# Autodesk Inventor assembly: Chassis-ver18-1111-2019
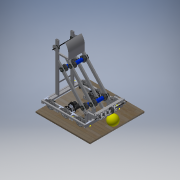
[picture p0: Inventor's stored thumbnail of the model, 180x180]
Saved by Autodesk Inventor 2018 (Build 220112000, 112)
## iProperties
Created: 2019-10-10
Part Number: Chassis-ver18-1111-2019
Document SubType Name: Assembly
Designer: JMHal
Author: JMHal
## Documents named in this file (21)
- F:\GrabCad\2020 Infinite Recharge\Chassis\Assembly\Chassis-ver18-1111-2019.iam
- F:\GrabCad\2020 Infinite Recharge\Chassis\Parts\2x1 20in Alluminum with Cal Drop.ver1-1111-2019.ipt
- F:\GrabCad\2020 Infinite Recharge\Chassis\Parts\2x1 20in Alluminum.ver1-1111-2019.ipt
- F:\GrabCad\2020 Infinite Recharge\Chassis\Parts\2x1 2in Alluminum Block.ver1-1111-2019.ipt
- F:\GrabCad\Resources\VEXpro Resources\Bearings\0.5inHexFlangedBearing(1.125inx0.313in)-1111-2016.ipt
- F:\GrabCad\Resources\VEXpro Resources\Versa Motion\VersaBlockKit-1111-2016.ipt
- F:\GrabCad\Resources\VEXpro Resources\Gearboxes\WCP SS Gearbox\SS-Gearbox.iam
- F:\GrabCad\Resources\VEXpro Resources\Gussets\ChassisGusset-1111-2016.ipt
- F:\GrabCad\Resources\VEXpro Resources\Wheels\6 inch\6x1inTractionWheel-1111-2016.iam
- F:\GrabCad\2020 Infinite Recharge\Chassis\Parts\Bumbers.ver1-1111-2019.ipt
- F:\GrabCad\Season Archives\2019 - Deep Space\Chassis\Parts\AluminumBracket.ipt
- F:\GrabCad\2020 Infinite Recharge\Chassis\Parts\BumperMount1-ver1-1111-2019.ipt
- F:\GrabCad\2020 Infinite Recharge\Intake\Assemblies\IntakeAssembly-ver1-1111-2020.iam
- F:\GrabCad\2020 Infinite Recharge\Platform.ver1-1111-2020.ipt
- F:\GrabCad\2020 Infinite Recharge\Powercell.ver1-1111-2020.ipt
- F:\GrabCad\2020 Infinite Recharge\Shooting\Assemblies\ShooterPrototype-ver2-1111-2019.iam
- F:\GrabCad\2020 Infinite Recharge\Storage\Assemblies\StorageAssembly.ver4-1111-2020.iam
- F:\GrabCad\2020 Infinite Recharge\Chassis\Parts\ElectricalBoard.ver2-1111-2020.ipt
- F:\GrabCad\Resources\VEXpro Resources\Shafts\0.5inThunderHexShaft(8)-1111-2016_MIR.ipt
- F:\GrabCad\Resources\VEXpro Resources\Shafts\0.5inThunderHexShaft(5in(modified))-1111-2016.ipt
- F:\GrabCad\2020 Infinite Recharge\Integration\Assemblies\Roller-ver1-1111-2019.iam
## Components (101 placed, 20 different names)
1. 2x1 20in Alluminum with Cal Drop.ver1-1111-2019:1 — Mate:31, Mate:32, Insert:8, Mate:53, Angle:9, Insert:19, Angle:11, Flush:1, Mate:65, Mate:66, Flush:2, Mate:67, Flush:4, Flush:5, Mate:77, Mate:78, Flush:16, Flush:17, Mate:80, Flush:20, Flush:23, Symmetry:1, Symmetry:2, Flush:62, Mate:141, Mate:146, Angle:15, Mate:147, Mate:148, Angle:16, Mate:149, Cylindrical:65, Mate:209, Angle:23, Mate:215, Flush:66, Mate:219, Flush:69
2. 2x1 20in Alluminum.ver1-1111-2019:1 — Mate:65, Mate:66, Flush:2, Mate:68, Mate:72, Mate:81, Flush:22, Mate:82, Flush:24, Flush:62, Mate:140, Flush:63, Mate:197, Mate:198, Mate:199, Mate:200, Mate:201, Mate:212
3. 2x1 20in Alluminum with Cal Drop.ver1-1111-2019:2 — Insert:5, Angle:7, Insert:23, Angle:13, Flush:6, Flush:8, Mate:73, Flush:9, Flush:34, Flush:35, Flush:36, Flush:37, Symmetry:1, Symmetry:2, Mate:142, Mate:143, Mate:156, Mate:157, Angle:17, Mate:158, Mate:159, Angle:18, Cylindrical:64, Mate:208, Angle:22, Mate:211, Flush:64, Flush:65
4. 2x1 20in Alluminum.ver1-1111-2019:2 — Mate:67, Flush:4, Flush:5, Mate:69, Flush:6, Mate:71, Mate:73, Mate:79, Flush:19, Flush:21, Mate:214, Flush:68
5. ChassisGusset-1111-2016:1 — Mate:76, Flush:12, Flush:36
6. ChassisGusset-1111-2016:2 — Mate:75, Flush:11, Flush:35
7. ChassisGusset-1111-2016:3 — Mate:78, Flush:14, Flush:17
8. ChassisGusset-1111-2016:4 — Mate:77, Flush:15, Flush:16
9. ChassisGusset-1111-2016:5 — Mate:82, Flush:24, Flush:34
10. ChassisGusset-1111-2016:6 — Mate:81, Flush:22, Flush:23
11. ChassisGusset-1111-2016:7 — Mate:80, Flush:20, Flush:21
12. ChassisGusset-1111-2016:8 — Mate:79, Flush:19, Flush:37, Mate:216
13. 6x1inTractionWheel-1111-2016:5 [sub-assembly] — Cylindrical:68, Mate:220
14. Bumbers.ver1-1111-2019:1 — Mate:139, Mate:140, Mate:210
15. VersaBlockKit-1111-2016:13 — Mate:146, Angle:15, Mate:147, Rotational:17
16. VersaBlockKit-1111-2016:14 — Mate:148, Angle:16, Mate:149, Cylindrical:45, Mate:153, Cylindrical:122, Mate:291
17. 0.5inHexFlangedBearing(1.125inx0.313in)-1111-2016:21 — Cylindrical:45, Mate:153
18. 6x1inTractionWheel-1111-2016:11 [sub-assembly] — Cylindrical:123, Mate:291
19. 0.5inHexFlangedBearing(1.125inx0.313in)-1111-2016:22 — Rotational:17
20. VersaBlockKit-1111-2016:15 — Mate:156, Mate:157, Angle:17, Mate:160, Angle:19, Mate:290
21. VersaBlockKit-1111-2016:16 — Mate:158, Mate:159, Angle:18, Mate:161, Mate:165, Angle:21
22. 0.5inHexFlangedBearing(1.125inx0.313in)-1111-2016:23 — Mate:160, Angle:19, Cylindrical:120
23. 0.5inHexFlangedBearing(1.125inx0.313in)-1111-2016:24 — Mate:161, Mate:165, Angle:21
24. 6x1inTractionWheel-1111-2016:12 [sub-assembly] — Cylindrical:121, Mate:290
25. 6x1inTractionWheel-1111-2016:13 [sub-assembly] — Cylindrical:124, Mate:292
26. 6x1inTractionWheel-1111-2016:14 [sub-assembly] — Cylindrical:69, Mate:221
27. AluminumBracket:1 — Mate:167, Mate:168, Mate:169
28. AluminumBracket:4 — Mate:176, Mate:177, Mate:178
29. AluminumBracket:5 — Mate:179, Mate:180, Mate:181
30. AluminumBracket:7 — Mate:185, Mate:186, Mate:187
31. BumperMount1-ver1-1111-2019:2 — Mate:197, Mate:198, Mate:199, Mate:210
32. BumperMount1-ver1-1111-2019:3 — Mate:200, Mate:201
33. SS-Gearbox:1 [sub-assembly] — Cylindrical:65, Mate:209, Angle:23, Cylindrical:124, Mate:292
34. SS-Gearbox:2 [sub-assembly] — Cylindrical:64, Mate:208, Angle:22, Cylindrical:69, Mate:221
35. IntakeAssembly-ver1-1111-2020:1 [sub-assembly] — Mate:211, Flush:64, Mate:212
36. Platform.ver1-1111-2020:1 — Flush:65, Mate:214, Tangent:2
37. Powercell.ver1-1111-2020:1 — Tangent:2
38. ShooterPrototype-ver2-1111-2019:1 [sub-assembly] — Mate:215, Flush:66, Mate:216, Mate:217, Flush:67, Mate:218
39. StorageAssembly.ver4-1111-2020:1 [sub-assembly] — Mate:217, Flush:67, Mate:218, Mate:234, Mate:235, Angle:24, Mate:237, Mate:238, Angle:25, Mate:241, Mate:242, Angle:26, Mate:243, Mate:244, Angle:27, Cylindrical:92, Mate:248, Mate:249, Angle:28, Mate:250, Mate:251, Angle:29, Mate:252, Mate:253, Angle:30, Mate:254, Mate:255, Angle:31, Mate:262, Mate:263, Angle:32, Mate:264, Mate:265, Angle:33, Mate:266, Mate:267, Angle:34, Mate:268, Mate:269, Angle:35, Mate:270, Mate:271, Angle:36, Mate:272, Mate:273, Angle:37, Mate:274, Mate:275, Angle:38, Mate:276, Mate:277, Angle:39
40. ElectricalBoard.ver2-1111-2020:1 — Mate:219, Flush:68, Flush:69
41. 0.5inThunderHexShaft(8)-1111-2016_MIR:1 — Cylindrical:67, Cylindrical:68
42. 0.5inThunderHexShaft(8)-1111-2016_MIR:2 — Cylindrical:120, Cylindrical:121
43. 0.5inHexFlangedBearing(1.125inx0.313in)-1111-2016:25 — Cylindrical:88, Mate:236, Flush:72
44. 0.5inHexFlangedBearing(1.125inx0.313in)-1111-2016:27 — Cylindrical:89, Mate:239, Cylindrical:90
45. 0.5inThunderHexShaft(5in(modified))-1111-2016:1 — Cylindrical:90, Flush:72
46. VersaBlockKit-1111-2016:17 — Mate:234, Mate:235, Angle:24, Cylindrical:88, Mate:236
47. VersaBlockKit-1111-2016:18 — Mate:237, Mate:238, Angle:25, Cylindrical:89, Mate:239
48. VersaBlockKit-1111-2016:19 — Mate:241, Mate:242, Angle:26, Mate:245
49. VersaBlockKit-1111-2016:20 — Mate:243, Mate:244, Angle:27, Cylindrical:93, Mate:246
50. 0.5inHexFlangedBearing(1.125inx0.313in)-1111-2016:33 — Cylindrical:92, Mate:245, Flush:73
51. 0.5inHexFlangedBearing(1.125inx0.313in)-1111-2016:34 — Cylindrical:93, Mate:246, Cylindrical:94
52. 0.5inThunderHexShaft(5in(modified))-1111-2016:5 — Cylindrical:94, Flush:73
53. VersaBlockKit-1111-2016:21 — Mate:248, Mate:249, Angle:28, Cylindrical:97, Mate:257
54. VersaBlockKit-1111-2016:22 — Mate:250, Mate:251, Angle:29, Cylindrical:96, Mate:256
55. VersaBlockKit-1111-2016:23 — Mate:252, Mate:253, Angle:30, Cylindrical:98, Mate:258
56. VersaBlockKit-1111-2016:24 — Mate:254, Mate:255, Angle:31, Cylindrical:99, Mate:259
57. 0.5inHexFlangedBearing(1.125inx0.313in)-1111-2016:35 — Cylindrical:96, Mate:256, Flush:70
58. 0.5inHexFlangedBearing(1.125inx0.313in)-1111-2016:36 — Cylindrical:97, Mate:257, Flush:71
59. 0.5inHexFlangedBearing(1.125inx0.313in)-1111-2016:37 — Cylindrical:98, Mate:258, Cylindrical:101
60. 0.5inHexFlangedBearing(1.125inx0.313in)-1111-2016:38 — Cylindrical:99, Mate:259, Cylindrical:100
61. 0.5inThunderHexShaft(5in(modified))-1111-2016:6 — Cylindrical:100, Flush:70
62. 0.5inThunderHexShaft(5in(modified))-1111-2016:7 — Cylindrical:101, Flush:71
63. VersaBlockKit-1111-2016:25 — Mate:262, Mate:263, Angle:32, Cylindrical:104, Mate:278
64. VersaBlockKit-1111-2016:26 — Mate:264, Mate:265, Angle:33, Cylindrical:105, Mate:279
65. VersaBlockKit-1111-2016:27 — Mate:266, Mate:267, Angle:34, Cylindrical:111, Mate:285
66. VersaBlockKit-1111-2016:28 — Mate:268, Mate:269, Angle:35, Cylindrical:109, Mate:283
67. VersaBlockKit-1111-2016:29 — Mate:270, Mate:271, Angle:36, Cylindrical:110, Mate:284
68. VersaBlockKit-1111-2016:30 — Mate:272, Mate:273, Angle:37, Cylindrical:108, Mate:282
69. VersaBlockKit-1111-2016:31 — Mate:274, Mate:275, Angle:38, Cylindrical:106, Mate:280
70. VersaBlockKit-1111-2016:32 — Mate:276, Mate:277, Angle:39, Cylindrical:107, Mate:281
71. 0.5inHexFlangedBearing(1.125inx0.313in)-1111-2016:39 — Cylindrical:104, Mate:278, Cylindrical:113, Flush:76
72. 0.5inHexFlangedBearing(1.125inx0.313in)-1111-2016:40 — Cylindrical:105, Mate:279, Cylindrical:115, Flush:75
73. 0.5inHexFlangedBearing(1.125inx0.313in)-1111-2016:41 — Cylindrical:106, Mate:280, Cylindrical:114, Flush:77
74. 0.5inHexFlangedBearing(1.125inx0.313in)-1111-2016:42 — Cylindrical:107, Mate:281, Cylindrical:112, Flush:74
75. 0.5inHexFlangedBearing(1.125inx0.313in)-1111-2016:43 — Cylindrical:108, Mate:282, Mate:305
76. 0.5inHexFlangedBearing(1.125inx0.313in)-1111-2016:44 — Cylindrical:109, Mate:283, Mate:306
77. 0.5inHexFlangedBearing(1.125inx0.313in)-1111-2016:45 — Cylindrical:110, Mate:284, Mate:307
78. 0.5inHexFlangedBearing(1.125inx0.313in)-1111-2016:46 — Cylindrical:111, Mate:285, Mate:308
79. 0.5inThunderHexShaft(5in(modified))-1111-2016:8 — Cylindrical:112, Cylindrical:138, Flush:74
80. 0.5inThunderHexShaft(5in(modified))-1111-2016:9 — Cylindrical:113, Cylindrical:137, Flush:76
81. 0.5inThunderHexShaft(5in(modified))-1111-2016:10 — Cylindrical:114, Cylindrical:136, Flush:77
82. 0.5inThunderHexShaft(5in(modified))-1111-2016:11 — Cylindrical:115, Cylindrical:139, Flush:75
83. 0.5inThunderHexShaft(8)-1111-2016_MIR:3 — Cylindrical:122, Cylindrical:123
84. 0.5inThunderHexShaft(8)-1111-2016_MIR:4 — Cylindrical:125, Cylindrical:126
85. 6x1inTractionWheel-1111-2016:15 [sub-assembly] — Cylindrical:126, Mate:293
86. Roller-ver1-1111-2019:1 [sub-assembly] — Cylindrical:136, Mate:305
87. Roller-ver1-1111-2019:2 [sub-assembly] — Cylindrical:137, Mate:306
88. Roller-ver1-1111-2019:3 [sub-assembly] — Cylindrical:138, Mate:307
89. Roller-ver1-1111-2019:4 [sub-assembly] — Cylindrical:139, Mate:308
90. 0.5inHexFlangedBearing(1.125inx0.313in)-1111-2016:19
91. 0.5inHexFlangedBearing(1.125inx0.313in)-1111-2016:7 — Insert:5, Mate:48, Mate:49
92. 0.5inHexFlangedBearing(1.125inx0.313in)-1111-2016:17 — Insert:19
93. 0.5inHexFlangedBearing(1.125inx0.313in)-1111-2016:10 — Insert:8, Mate:52, Cylindrical:125
94. 2x1 2in Alluminum Block.ver1-1111-2019:5 — Mate:31, Mate:32, Mate:69, Flush:15, Mate:167, Mate:168, Mate:169
95. 2x1 2in Alluminum Block.ver1-1111-2019:6 — Flush:1, Mate:68, Flush:14, Mate:141, Mate:176, Mate:177, Mate:178
96. 2x1 2in Alluminum Block.ver1-1111-2019:7 — Mate:72, Flush:9, Mate:75, Flush:11, Mate:143, Flush:63, Mate:179, Mate:180, Mate:181
97. 2x1 2in Alluminum Block.ver1-1111-2019:8 — Flush:8, Mate:71, Mate:76, Flush:12, Mate:139, Mate:142, Mate:185, Mate:186, Mate:187
98. VersaBlockKit-1111-2016:3 — Mate:48, Mate:49, Angle:7, Cylindrical:67, Mate:220
99. VersaBlockKit-1111-2016:6 — Mate:52, Mate:53, Angle:9, Mate:293
100. VersaBlockKit-1111-2016:9 — Angle:11
101. VersaBlockKit-1111-2016:11 — Insert:23, Angle:13
## Relationships (245: Mate 127, CylindricalJoint 41, Flush 39, Angle 28, Insert 6, Symmetry 2, RevoluteJoint 1, Tangent 1)
- Mate:31: 2x1 20in Alluminum with Cal Drop.ver1-1111-2019:1 ↔ 2x1 2in Alluminum Block.ver1-1111-2019:5
- Mate:32: 2x1 20in Alluminum with Cal Drop.ver1-1111-2019:1 ↔ 2x1 2in Alluminum Block.ver1-1111-2019:5
- Insert:5: 2x1 20in Alluminum with Cal Drop.ver1-1111-2019:2 ↔ 0.5inHexFlangedBearing(1.125inx0.313in)-1111-2016:7
- Mate:48: 0.5inHexFlangedBearing(1.125inx0.313in)-1111-2016:7 ↔ VersaBlockKit-1111-2016:3
- Mate:49: 0.5inHexFlangedBearing(1.125inx0.313in)-1111-2016:7 ↔ VersaBlockKit-1111-2016:3
- Insert:8: 2x1 20in Alluminum with Cal Drop.ver1-1111-2019:1 ↔ 0.5inHexFlangedBearing(1.125inx0.313in)-1111-2016:10
- Angle:7 (0 deg): 2x1 20in Alluminum with Cal Drop.ver1-1111-2019:2 ↔ VersaBlockKit-1111-2016:3
- Mate:52: 0.5inHexFlangedBearing(1.125inx0.313in)-1111-2016:10 ↔ VersaBlockKit-1111-2016:6
- Mate:53: 2x1 20in Alluminum with Cal Drop.ver1-1111-2019:1 ↔ VersaBlockKit-1111-2016:6
- Angle:9 (0 deg): 2x1 20in Alluminum with Cal Drop.ver1-1111-2019:1 ↔ VersaBlockKit-1111-2016:6
- [Mate]: 0.5inHexFlangedBearing(1.125inx0.313in)-1111-2016:17 ↔ VersaBlockKit-1111-2016:9
- [Insert]: 0.5inHexFlangedBearing(1.125inx0.313in)-1111-2016:17 ↔ VersaBlockKit-1111-2016:9
- Insert:19: 2x1 20in Alluminum with Cal Drop.ver1-1111-2019:1 ↔ 0.5inHexFlangedBearing(1.125inx0.313in)-1111-2016:17
- Angle:11 (0 deg): 2x1 20in Alluminum with Cal Drop.ver1-1111-2019:1 ↔ VersaBlockKit-1111-2016:9
- [Mate]: 0.5inHexFlangedBearing(1.125inx0.313in)-1111-2016:19 ↔ VersaBlockKit-1111-2016:11
- [Insert]: 0.5inHexFlangedBearing(1.125inx0.313in)-1111-2016:19 ↔ VersaBlockKit-1111-2016:11
- Insert:23: 2x1 20in Alluminum with Cal Drop.ver1-1111-2019:2 ↔ VersaBlockKit-1111-2016:11
- Angle:13 (0 deg): 2x1 20in Alluminum with Cal Drop.ver1-1111-2019:2 ↔ VersaBlockKit-1111-2016:11
- Flush:1: 2x1 20in Alluminum with Cal Drop.ver1-1111-2019:1 ↔ 2x1 2in Alluminum Block.ver1-1111-2019:6
- Mate:65: 2x1 20in Alluminum with Cal Drop.ver1-1111-2019:1 ↔ 2x1 20in Alluminum.ver1-1111-2019:1
- Mate:66: 2x1 20in Alluminum with Cal Drop.ver1-1111-2019:1 ↔ 2x1 20in Alluminum.ver1-1111-2019:1
- Flush:2: 2x1 20in Alluminum with Cal Drop.ver1-1111-2019:1 ↔ 2x1 20in Alluminum.ver1-1111-2019:1
- Mate:67: 2x1 20in Alluminum with Cal Drop.ver1-1111-2019:1 ↔ 2x1 20in Alluminum.ver1-1111-2019:2
- Flush:4: 2x1 20in Alluminum with Cal Drop.ver1-1111-2019:1 ↔ 2x1 20in Alluminum.ver1-1111-2019:2
- Flush:5 (-69.85 mm): 2x1 20in Alluminum with Cal Drop.ver1-1111-2019:1 ↔ 2x1 20in Alluminum.ver1-1111-2019:2
- Mate:68 (254 mm): 2x1 20in Alluminum.ver1-1111-2019:1 ↔ 2x1 2in Alluminum Block.ver1-1111-2019:6
- Mate:69 (254 mm): 2x1 20in Alluminum.ver1-1111-2019:2 ↔ 2x1 2in Alluminum Block.ver1-1111-2019:5
- Flush:6: 2x1 20in Alluminum with Cal Drop.ver1-1111-2019:2 ↔ 2x1 20in Alluminum.ver1-1111-2019:2
- Flush:8: 2x1 20in Alluminum with Cal Drop.ver1-1111-2019:2 ↔ 2x1 2in Alluminum Block.ver1-1111-2019:8
- Mate:71 (254 mm): 2x1 20in Alluminum.ver1-1111-2019:2 ↔ 2x1 2in Alluminum Block.ver1-1111-2019:8
- Mate:72 (254 mm): 2x1 20in Alluminum.ver1-1111-2019:1 ↔ 2x1 2in Alluminum Block.ver1-1111-2019:7
- Mate:73: 2x1 20in Alluminum with Cal Drop.ver1-1111-2019:2 ↔ 2x1 20in Alluminum.ver1-1111-2019:2
- Flush:9: 2x1 20in Alluminum with Cal Drop.ver1-1111-2019:2 ↔ 2x1 2in Alluminum Block.ver1-1111-2019:7
- Mate:75: ChassisGusset-1111-2016:2 ↔ 2x1 2in Alluminum Block.ver1-1111-2019:7
- Flush:11: ChassisGusset-1111-2016:2 ↔ 2x1 2in Alluminum Block.ver1-1111-2019:7
- Mate:76: ChassisGusset-1111-2016:1 ↔ 2x1 2in Alluminum Block.ver1-1111-2019:8
- Flush:12: ChassisGusset-1111-2016:1 ↔ 2x1 2in Alluminum Block.ver1-1111-2019:8
- Mate:77: 2x1 20in Alluminum with Cal Drop.ver1-1111-2019:1 ↔ ChassisGusset-1111-2016:4
- Mate:78: 2x1 20in Alluminum with Cal Drop.ver1-1111-2019:1 ↔ ChassisGusset-1111-2016:3
- Flush:14: ChassisGusset-1111-2016:3 ↔ 2x1 2in Alluminum Block.ver1-1111-2019:6
- Flush:15: ChassisGusset-1111-2016:4 ↔ 2x1 2in Alluminum Block.ver1-1111-2019:5
- Flush:16: 2x1 20in Alluminum with Cal Drop.ver1-1111-2019:1 ↔ ChassisGusset-1111-2016:4
- Flush:17: 2x1 20in Alluminum with Cal Drop.ver1-1111-2019:1 ↔ ChassisGusset-1111-2016:3
- Mate:79: 2x1 20in Alluminum.ver1-1111-2019:2 ↔ ChassisGusset-1111-2016:8
- Flush:19: 2x1 20in Alluminum.ver1-1111-2019:2 ↔ ChassisGusset-1111-2016:8
- Mate:80: 2x1 20in Alluminum with Cal Drop.ver1-1111-2019:1 ↔ ChassisGusset-1111-2016:7
- Flush:20: 2x1 20in Alluminum with Cal Drop.ver1-1111-2019:1 ↔ ChassisGusset-1111-2016:7
- Flush:21: 2x1 20in Alluminum.ver1-1111-2019:2 ↔ ChassisGusset-1111-2016:7
- Mate:81: 2x1 20in Alluminum.ver1-1111-2019:1 ↔ ChassisGusset-1111-2016:6
- Flush:22: 2x1 20in Alluminum.ver1-1111-2019:1 ↔ ChassisGusset-1111-2016:6
- Flush:23: 2x1 20in Alluminum with Cal Drop.ver1-1111-2019:1 ↔ ChassisGusset-1111-2016:6
- Mate:82: 2x1 20in Alluminum.ver1-1111-2019:1 ↔ ChassisGusset-1111-2016:5
- Flush:24: 2x1 20in Alluminum.ver1-1111-2019:1 ↔ ChassisGusset-1111-2016:5
- Flush:34: 2x1 20in Alluminum with Cal Drop.ver1-1111-2019:2 ↔ ChassisGusset-1111-2016:5
- Flush:35: 2x1 20in Alluminum with Cal Drop.ver1-1111-2019:2 ↔ ChassisGusset-1111-2016:2
- Flush:36: 2x1 20in Alluminum with Cal Drop.ver1-1111-2019:2 ↔ ChassisGusset-1111-2016:1
- Flush:37: 2x1 20in Alluminum with Cal Drop.ver1-1111-2019:2 ↔ ChassisGusset-1111-2016:8
- Symmetry:1: 2x1 20in Alluminum with Cal Drop.ver1-1111-2019:1 ↔ 2x1 20in Alluminum with Cal Drop.ver1-1111-2019:2
- Symmetry:2: 2x1 20in Alluminum with Cal Drop.ver1-1111-2019:1 ↔ 2x1 20in Alluminum with Cal Drop.ver1-1111-2019:2
- Flush:62 (69.85 mm): 2x1 20in Alluminum with Cal Drop.ver1-1111-2019:1 ↔ 2x1 20in Alluminum.ver1-1111-2019:1
- Mate:139 (-127 mm): Bumbers.ver1-1111-2019:1 ↔ 2x1 2in Alluminum Block.ver1-1111-2019:8
- Mate:140: 2x1 20in Alluminum.ver1-1111-2019:1 ↔ Bumbers.ver1-1111-2019:1
- Mate:141: 2x1 20in Alluminum with Cal Drop.ver1-1111-2019:1 ↔ 2x1 2in Alluminum Block.ver1-1111-2019:6
- Mate:142: 2x1 20in Alluminum with Cal Drop.ver1-1111-2019:2 ↔ 2x1 2in Alluminum Block.ver1-1111-2019:8
- Mate:143: 2x1 20in Alluminum with Cal Drop.ver1-1111-2019:2 ↔ 2x1 2in Alluminum Block.ver1-1111-2019:7
- Flush:63: 2x1 20in Alluminum.ver1-1111-2019:1 ↔ 2x1 2in Alluminum Block.ver1-1111-2019:7
- Mate:146: 2x1 20in Alluminum with Cal Drop.ver1-1111-2019:1 ↔ VersaBlockKit-1111-2016:13
- Angle:15 (0 deg): 2x1 20in Alluminum with Cal Drop.ver1-1111-2019:1 ↔ VersaBlockKit-1111-2016:13
- Mate:147: 2x1 20in Alluminum with Cal Drop.ver1-1111-2019:1 ↔ VersaBlockKit-1111-2016:13
- Mate:148: 2x1 20in Alluminum with Cal Drop.ver1-1111-2019:1 ↔ VersaBlockKit-1111-2016:14
- Angle:16 (0 deg): 2x1 20in Alluminum with Cal Drop.ver1-1111-2019:1 ↔ VersaBlockKit-1111-2016:14
- Mate:149: 2x1 20in Alluminum with Cal Drop.ver1-1111-2019:1 ↔ VersaBlockKit-1111-2016:14
- Cylindrical:45: VersaBlockKit-1111-2016:14 ↔ 0.5inHexFlangedBearing(1.125inx0.313in)-1111-2016:21
- Rotational:17 [RevoluteJoint]: VersaBlockKit-1111-2016:13 ↔ 0.5inHexFlangedBearing(1.125inx0.313in)-1111-2016:22
- Mate:153: VersaBlockKit-1111-2016:14 ↔ 0.5inHexFlangedBearing(1.125inx0.313in)-1111-2016:21
- Mate:156: 2x1 20in Alluminum with Cal Drop.ver1-1111-2019:2 ↔ VersaBlockKit-1111-2016:15
- Mate:157: 2x1 20in Alluminum with Cal Drop.ver1-1111-2019:2 ↔ VersaBlockKit-1111-2016:15
- Angle:17 (0 deg): 2x1 20in Alluminum with Cal Drop.ver1-1111-2019:2 ↔ VersaBlockKit-1111-2016:15
- Mate:158: 2x1 20in Alluminum with Cal Drop.ver1-1111-2019:2 ↔ VersaBlockKit-1111-2016:16
- Mate:159: 2x1 20in Alluminum with Cal Drop.ver1-1111-2019:2 ↔ VersaBlockKit-1111-2016:16
- Angle:18 (0 deg): 2x1 20in Alluminum with Cal Drop.ver1-1111-2019:2 ↔ VersaBlockKit-1111-2016:16
- Mate:160: VersaBlockKit-1111-2016:15 ↔ 0.5inHexFlangedBearing(1.125inx0.313in)-1111-2016:23
- Mate:161: VersaBlockKit-1111-2016:16 ↔ 0.5inHexFlangedBearing(1.125inx0.313in)-1111-2016:24
- Angle:19 (0 deg): VersaBlockKit-1111-2016:15 ↔ 0.5inHexFlangedBearing(1.125inx0.313in)-1111-2016:23
- Mate:165: VersaBlockKit-1111-2016:16 ↔ 0.5inHexFlangedBearing(1.125inx0.313in)-1111-2016:24
- Angle:21 (0 deg): VersaBlockKit-1111-2016:16 ↔ 0.5inHexFlangedBearing(1.125inx0.313in)-1111-2016:24
- Mate:167: AluminumBracket:1 ↔ 2x1 2in Alluminum Block.ver1-1111-2019:5
- Mate:168: AluminumBracket:1 ↔ 2x1 2in Alluminum Block.ver1-1111-2019:5
- Mate:169: AluminumBracket:1 ↔ 2x1 2in Alluminum Block.ver1-1111-2019:5
- Mate:176: AluminumBracket:4 ↔ 2x1 2in Alluminum Block.ver1-1111-2019:6
- Mate:177: AluminumBracket:4 ↔ 2x1 2in Alluminum Block.ver1-1111-2019:6
- Mate:178 (0.127 mm): AluminumBracket:4 ↔ 2x1 2in Alluminum Block.ver1-1111-2019:6
- Mate:179: AluminumBracket:5 ↔ 2x1 2in Alluminum Block.ver1-1111-2019:7
- Mate:180: AluminumBracket:5 ↔ 2x1 2in Alluminum Block.ver1-1111-2019:7
- Mate:181 (0.0762 mm): AluminumBracket:5 ↔ 2x1 2in Alluminum Block.ver1-1111-2019:7
- Mate:185: AluminumBracket:7 ↔ 2x1 2in Alluminum Block.ver1-1111-2019:8
- Mate:186: AluminumBracket:7 ↔ 2x1 2in Alluminum Block.ver1-1111-2019:8
- Mate:187 (0.6096 mm): AluminumBracket:7 ↔ 2x1 2in Alluminum Block.ver1-1111-2019:8
- Mate:197: 2x1 20in Alluminum.ver1-1111-2019:1 ↔ BumperMount1-ver1-1111-2019:2
- Mate:198: 2x1 20in Alluminum.ver1-1111-2019:1 ↔ BumperMount1-ver1-1111-2019:2
- Mate:199: 2x1 20in Alluminum.ver1-1111-2019:1 ↔ BumperMount1-ver1-1111-2019:2
- Mate:200: 2x1 20in Alluminum.ver1-1111-2019:1 ↔ BumperMount1-ver1-1111-2019:3
- Mate:201: 2x1 20in Alluminum.ver1-1111-2019:1 ↔ BumperMount1-ver1-1111-2019:3
- Cylindrical:64: 2x1 20in Alluminum with Cal Drop.ver1-1111-2019:2 ↔ SS-Gearbox:2
- Mate:208: 2x1 20in Alluminum with Cal Drop.ver1-1111-2019:2 ↔ SS-Gearbox:2
- Angle:22 (90 deg): 2x1 20in Alluminum with Cal Drop.ver1-1111-2019:2 ↔ SS-Gearbox:2
- Cylindrical:65: 2x1 20in Alluminum with Cal Drop.ver1-1111-2019:1 ↔ SS-Gearbox:1
- Mate:209: 2x1 20in Alluminum with Cal Drop.ver1-1111-2019:1 ↔ SS-Gearbox:1
- Angle:23 (-90 deg): 2x1 20in Alluminum with Cal Drop.ver1-1111-2019:1 ↔ SS-Gearbox:1
- Mate:210: Bumbers.ver1-1111-2019:1 ↔ BumperMount1-ver1-1111-2019:2
- Mate:211: 2x1 20in Alluminum with Cal Drop.ver1-1111-2019:2 ↔ IntakeAssembly-ver1-1111-2020:1
- Flush:64 (-8.3185 mm): 2x1 20in Alluminum with Cal Drop.ver1-1111-2019:2 ↔ IntakeAssembly-ver1-1111-2020:1
- Mate:212: 2x1 20in Alluminum.ver1-1111-2019:1 ↔ IntakeAssembly-ver1-1111-2020:1
- Flush:65 (-203.2 mm): 2x1 20in Alluminum with Cal Drop.ver1-1111-2019:2 ↔ Platform.ver1-1111-2020:1
- Mate:214: 2x1 20in Alluminum.ver1-1111-2019:2 ↔ Platform.ver1-1111-2020:1
- Mate:215: 2x1 20in Alluminum with Cal Drop.ver1-1111-2019:1 ↔ ShooterPrototype-ver2-1111-2019:1
- Flush:66: 2x1 20in Alluminum with Cal Drop.ver1-1111-2019:1 ↔ ShooterPrototype-ver2-1111-2019:1
- Mate:216: ChassisGusset-1111-2016:8 ↔ ShooterPrototype-ver2-1111-2019:1
- Mate:217: ShooterPrototype-ver2-1111-2019:1 ↔ StorageAssembly.ver4-1111-2020:1
- Flush:67: ShooterPrototype-ver2-1111-2019:1 ↔ StorageAssembly.ver4-1111-2020:1
- Mate:218: ShooterPrototype-ver2-1111-2019:1 ↔ StorageAssembly.ver4-1111-2020:1
- Mate:219: 2x1 20in Alluminum with Cal Drop.ver1-1111-2019:1 ↔ ElectricalBoard.ver2-1111-2020:1
- Flush:68: 2x1 20in Alluminum.ver1-1111-2019:2 ↔ ElectricalBoard.ver2-1111-2020:1
- Flush:69: 2x1 20in Alluminum with Cal Drop.ver1-1111-2019:1 ↔ ElectricalBoard.ver2-1111-2020:1
- Tangent:2: Platform.ver1-1111-2020:1 ↔ Powercell.ver1-1111-2020:1
- Cylindrical:67: 0.5inThunderHexShaft(8)-1111-2016_MIR:1 ↔ VersaBlockKit-1111-2016:3
- Cylindrical:68: 6x1inTractionWheel-1111-2016:5 ↔ 0.5inThunderHexShaft(8)-1111-2016_MIR:1
- Mate:220 (6.35 mm): 6x1inTractionWheel-1111-2016:5 ↔ VersaBlockKit-1111-2016:3
- Cylindrical:69: 6x1inTractionWheel-1111-2016:14 ↔ SS-Gearbox:2
- Mate:221 (6.35 mm): 6x1inTractionWheel-1111-2016:14 ↔ SS-Gearbox:2
- Mate:234: StorageAssembly.ver4-1111-2020:1 ↔ VersaBlockKit-1111-2016:17
- Mate:235: StorageAssembly.ver4-1111-2020:1 ↔ VersaBlockKit-1111-2016:17
- Angle:24 (0 deg): StorageAssembly.ver4-1111-2020:1 ↔ VersaBlockKit-1111-2016:17
- Cylindrical:88: 0.5inHexFlangedBearing(1.125inx0.313in)-1111-2016:25 ↔ VersaBlockKit-1111-2016:17
- Mate:236: 0.5inHexFlangedBearing(1.125inx0.313in)-1111-2016:25 ↔ VersaBlockKit-1111-2016:17
- Mate:237: StorageAssembly.ver4-1111-2020:1 ↔ VersaBlockKit-1111-2016:18
- Mate:238: StorageAssembly.ver4-1111-2020:1 ↔ VersaBlockKit-1111-2016:18
- Angle:25 (0 deg): StorageAssembly.ver4-1111-2020:1 ↔ VersaBlockKit-1111-2016:18
- Cylindrical:89: 0.5inHexFlangedBearing(1.125inx0.313in)-1111-2016:27 ↔ VersaBlockKit-1111-2016:18
- Mate:239: 0.5inHexFlangedBearing(1.125inx0.313in)-1111-2016:27 ↔ VersaBlockKit-1111-2016:18
- Cylindrical:90: 0.5inHexFlangedBearing(1.125inx0.313in)-1111-2016:27 ↔ 0.5inThunderHexShaft(5in(modified))-1111-2016:1
- Mate:241: StorageAssembly.ver4-1111-2020:1 ↔ VersaBlockKit-1111-2016:19
- Mate:242: StorageAssembly.ver4-1111-2020:1 ↔ VersaBlockKit-1111-2016:19
- Angle:26 (0 deg): StorageAssembly.ver4-1111-2020:1 ↔ VersaBlockKit-1111-2016:19
- Mate:243: StorageAssembly.ver4-1111-2020:1 ↔ VersaBlockKit-1111-2016:20
- Mate:244: StorageAssembly.ver4-1111-2020:1 ↔ VersaBlockKit-1111-2016:20
- Angle:27 (0 deg): StorageAssembly.ver4-1111-2020:1 ↔ VersaBlockKit-1111-2016:20
- Cylindrical:92: StorageAssembly.ver4-1111-2020:1 ↔ 0.5inHexFlangedBearing(1.125inx0.313in)-1111-2016:33
- Mate:245: VersaBlockKit-1111-2016:19 ↔ 0.5inHexFlangedBearing(1.125inx0.313in)-1111-2016:33
- Cylindrical:93: VersaBlockKit-1111-2016:20 ↔ 0.5inHexFlangedBearing(1.125inx0.313in)-1111-2016:34
- Mate:246: VersaBlockKit-1111-2016:20 ↔ 0.5inHexFlangedBearing(1.125inx0.313in)-1111-2016:34
- Cylindrical:94: 0.5inHexFlangedBearing(1.125inx0.313in)-1111-2016:34 ↔ 0.5inThunderHexShaft(5in(modified))-1111-2016:5
- Mate:248: StorageAssembly.ver4-1111-2020:1 ↔ VersaBlockKit-1111-2016:21
- Mate:249: StorageAssembly.ver4-1111-2020:1 ↔ VersaBlockKit-1111-2016:21
- Angle:28 (0 deg): StorageAssembly.ver4-1111-2020:1 ↔ VersaBlockKit-1111-2016:21
- Mate:250: StorageAssembly.ver4-1111-2020:1 ↔ VersaBlockKit-1111-2016:22
- Mate:251: StorageAssembly.ver4-1111-2020:1 ↔ VersaBlockKit-1111-2016:22
- Angle:29 (0 deg): StorageAssembly.ver4-1111-2020:1 ↔ VersaBlockKit-1111-2016:22
- Mate:252: StorageAssembly.ver4-1111-2020:1 ↔ VersaBlockKit-1111-2016:23
- Mate:253: StorageAssembly.ver4-1111-2020:1 ↔ VersaBlockKit-1111-2016:23
- Angle:30 (0 deg): StorageAssembly.ver4-1111-2020:1 ↔ VersaBlockKit-1111-2016:23
- Mate:254: StorageAssembly.ver4-1111-2020:1 ↔ VersaBlockKit-1111-2016:24
- Mate:255: StorageAssembly.ver4-1111-2020:1 ↔ VersaBlockKit-1111-2016:24
- Angle:31 (0 deg): StorageAssembly.ver4-1111-2020:1 ↔ VersaBlockKit-1111-2016:24
- Cylindrical:96: VersaBlockKit-1111-2016:22 ↔ 0.5inHexFlangedBearing(1.125inx0.313in)-1111-2016:35
- Mate:256: VersaBlockKit-1111-2016:22 ↔ 0.5inHexFlangedBearing(1.125inx0.313in)-1111-2016:35
- Cylindrical:97: VersaBlockKit-1111-2016:21 ↔ 0.5inHexFlangedBearing(1.125inx0.313in)-1111-2016:36
- Mate:257: VersaBlockKit-1111-2016:21 ↔ 0.5inHexFlangedBearing(1.125inx0.313in)-1111-2016:36
- Cylindrical:98: VersaBlockKit-1111-2016:23 ↔ 0.5inHexFlangedBearing(1.125inx0.313in)-1111-2016:37
- Mate:258: VersaBlockKit-1111-2016:23 ↔ 0.5inHexFlangedBearing(1.125inx0.313in)-1111-2016:37
- Cylindrical:99: VersaBlockKit-1111-2016:24 ↔ 0.5inHexFlangedBearing(1.125inx0.313in)-1111-2016:38
- Mate:259: VersaBlockKit-1111-2016:24 ↔ 0.5inHexFlangedBearing(1.125inx0.313in)-1111-2016:38
- Cylindrical:100: 0.5inHexFlangedBearing(1.125inx0.313in)-1111-2016:38 ↔ 0.5inThunderHexShaft(5in(modified))-1111-2016:6
- Cylindrical:101: 0.5inHexFlangedBearing(1.125inx0.313in)-1111-2016:37 ↔ 0.5inThunderHexShaft(5in(modified))-1111-2016:7
- Mate:262: StorageAssembly.ver4-1111-2020:1 ↔ VersaBlockKit-1111-2016:25
- Mate:263: StorageAssembly.ver4-1111-2020:1 ↔ VersaBlockKit-1111-2016:25
- Angle:32 (0 deg): StorageAssembly.ver4-1111-2020:1 ↔ VersaBlockKit-1111-2016:25
- Mate:264: StorageAssembly.ver4-1111-2020:1 ↔ VersaBlockKit-1111-2016:26
- Mate:265: StorageAssembly.ver4-1111-2020:1 ↔ VersaBlockKit-1111-2016:26
- Angle:33 (0 deg): StorageAssembly.ver4-1111-2020:1 ↔ VersaBlockKit-1111-2016:26
- Mate:266: StorageAssembly.ver4-1111-2020:1 ↔ VersaBlockKit-1111-2016:27
- Mate:267: StorageAssembly.ver4-1111-2020:1 ↔ VersaBlockKit-1111-2016:27
- Angle:34 (0 deg): StorageAssembly.ver4-1111-2020:1 ↔ VersaBlockKit-1111-2016:27
- Mate:268: StorageAssembly.ver4-1111-2020:1 ↔ VersaBlockKit-1111-2016:28
- Mate:269: StorageAssembly.ver4-1111-2020:1 ↔ VersaBlockKit-1111-2016:28
- Angle:35 (0 deg): StorageAssembly.ver4-1111-2020:1 ↔ VersaBlockKit-1111-2016:28
- Mate:270: StorageAssembly.ver4-1111-2020:1 ↔ VersaBlockKit-1111-2016:29
- Mate:271: StorageAssembly.ver4-1111-2020:1 ↔ VersaBlockKit-1111-2016:29
- Angle:36 (0 deg): StorageAssembly.ver4-1111-2020:1 ↔ VersaBlockKit-1111-2016:29
- Mate:272: StorageAssembly.ver4-1111-2020:1 ↔ VersaBlockKit-1111-2016:30
- Mate:273: StorageAssembly.ver4-1111-2020:1 ↔ VersaBlockKit-1111-2016:30
- Angle:37 (0 deg): StorageAssembly.ver4-1111-2020:1 ↔ VersaBlockKit-1111-2016:30
- Mate:274: StorageAssembly.ver4-1111-2020:1 ↔ VersaBlockKit-1111-2016:31
- Mate:275: StorageAssembly.ver4-1111-2020:1 ↔ VersaBlockKit-1111-2016:31
- Angle:38 (0 deg): StorageAssembly.ver4-1111-2020:1 ↔ VersaBlockKit-1111-2016:31
- Mate:276: StorageAssembly.ver4-1111-2020:1 ↔ VersaBlockKit-1111-2016:32
- Mate:277: StorageAssembly.ver4-1111-2020:1 ↔ VersaBlockKit-1111-2016:32
- Angle:39 (0 deg): StorageAssembly.ver4-1111-2020:1 ↔ VersaBlockKit-1111-2016:32
- Cylindrical:104: VersaBlockKit-1111-2016:25 ↔ 0.5inHexFlangedBearing(1.125inx0.313in)-1111-2016:39
- Mate:278: VersaBlockKit-1111-2016:25 ↔ 0.5inHexFlangedBearing(1.125inx0.313in)-1111-2016:39
- Cylindrical:105: VersaBlockKit-1111-2016:26 ↔ 0.5inHexFlangedBearing(1.125inx0.313in)-1111-2016:40
- Mate:279: VersaBlockKit-1111-2016:26 ↔ 0.5inHexFlangedBearing(1.125inx0.313in)-1111-2016:40
- Cylindrical:106: VersaBlockKit-1111-2016:31 ↔ 0.5inHexFlangedBearing(1.125inx0.313in)-1111-2016:41
- Mate:280: VersaBlockKit-1111-2016:31 ↔ 0.5inHexFlangedBearing(1.125inx0.313in)-1111-2016:41
- Cylindrical:107: VersaBlockKit-1111-2016:32 ↔ 0.5inHexFlangedBearing(1.125inx0.313in)-1111-2016:42
- Mate:281: VersaBlockKit-1111-2016:32 ↔ 0.5inHexFlangedBearing(1.125inx0.313in)-1111-2016:42
- Cylindrical:108: VersaBlockKit-1111-2016:30 ↔ 0.5inHexFlangedBearing(1.125inx0.313in)-1111-2016:43
- Mate:282: VersaBlockKit-1111-2016:30 ↔ 0.5inHexFlangedBearing(1.125inx0.313in)-1111-2016:43
- Cylindrical:109: VersaBlockKit-1111-2016:28 ↔ 0.5inHexFlangedBearing(1.125inx0.313in)-1111-2016:44
- Mate:283: VersaBlockKit-1111-2016:28 ↔ 0.5inHexFlangedBearing(1.125inx0.313in)-1111-2016:44
- Cylindrical:110: VersaBlockKit-1111-2016:29 ↔ 0.5inHexFlangedBearing(1.125inx0.313in)-1111-2016:45
- Mate:284: VersaBlockKit-1111-2016:29 ↔ 0.5inHexFlangedBearing(1.125inx0.313in)-1111-2016:45
- Cylindrical:111: VersaBlockKit-1111-2016:27 ↔ 0.5inHexFlangedBearing(1.125inx0.313in)-1111-2016:46
- Mate:285: VersaBlockKit-1111-2016:27 ↔ 0.5inHexFlangedBearing(1.125inx0.313in)-1111-2016:46
- Cylindrical:112: 0.5inHexFlangedBearing(1.125inx0.313in)-1111-2016:42 ↔ 0.5inThunderHexShaft(5in(modified))-1111-2016:8
- Cylindrical:113: 0.5inHexFlangedBearing(1.125inx0.313in)-1111-2016:39 ↔ 0.5inThunderHexShaft(5in(modified))-1111-2016:9
- Cylindrical:114: 0.5inHexFlangedBearing(1.125inx0.313in)-1111-2016:41 ↔ 0.5inThunderHexShaft(5in(modified))-1111-2016:10
- Cylindrical:115: 0.5inHexFlangedBearing(1.125inx0.313in)-1111-2016:40 ↔ 0.5inThunderHexShaft(5in(modified))-1111-2016:11
- Cylindrical:120: 0.5inHexFlangedBearing(1.125inx0.313in)-1111-2016:23 ↔ 0.5inThunderHexShaft(8)-1111-2016_MIR:2
- Cylindrical:121: 6x1inTractionWheel-1111-2016:12 ↔ 0.5inThunderHexShaft(8)-1111-2016_MIR:2
- Mate:290 (6.35 mm): VersaBlockKit-1111-2016:15 ↔ 6x1inTractionWheel-1111-2016:12
- Cylindrical:122: VersaBlockKit-1111-2016:14 ↔ 0.5inThunderHexShaft(8)-1111-2016_MIR:3
- Cylindrical:123: 6x1inTractionWheel-1111-2016:11 ↔ 0.5inThunderHexShaft(8)-1111-2016_MIR:3
- Mate:291 (6.35 mm): VersaBlockKit-1111-2016:14 ↔ 6x1inTractionWheel-1111-2016:11
- Cylindrical:124: 6x1inTractionWheel-1111-2016:13 ↔ SS-Gearbox:1
- Mate:292 (6.35 mm): 6x1inTractionWheel-1111-2016:13 ↔ SS-Gearbox:1
- Cylindrical:125: 0.5inThunderHexShaft(8)-1111-2016_MIR:4 ↔ 0.5inHexFlangedBearing(1.125inx0.313in)-1111-2016:10
- Cylindrical:126: 0.5inThunderHexShaft(8)-1111-2016_MIR:4 ↔ 6x1inTractionWheel-1111-2016:15
- Mate:293 (6.35 mm): 6x1inTractionWheel-1111-2016:15 ↔ VersaBlockKit-1111-2016:6
- Cylindrical:136: 0.5inThunderHexShaft(5in(modified))-1111-2016:10 ↔ Roller-ver1-1111-2019:1
- Mate:305 (11.1125 mm): 0.5inHexFlangedBearing(1.125inx0.313in)-1111-2016:43 ↔ Roller-ver1-1111-2019:1
- Cylindrical:137: 0.5inThunderHexShaft(5in(modified))-1111-2016:9 ↔ Roller-ver1-1111-2019:2
- Mate:306 (11.1125 mm): 0.5inHexFlangedBearing(1.125inx0.313in)-1111-2016:44 ↔ Roller-ver1-1111-2019:2
- Cylindrical:138: 0.5inThunderHexShaft(5in(modified))-1111-2016:8 ↔ Roller-ver1-1111-2019:3
- Mate:307 (11.1125 mm): 0.5inHexFlangedBearing(1.125inx0.313in)-1111-2016:45 ↔ Roller-ver1-1111-2019:3
- Cylindrical:139: 0.5inThunderHexShaft(5in(modified))-1111-2016:11 ↔ Roller-ver1-1111-2019:4
- Mate:308 (11.1125 mm): 0.5inHexFlangedBearing(1.125inx0.313in)-1111-2016:46 ↔ Roller-ver1-1111-2019:4
- Flush:70: 0.5inHexFlangedBearing(1.125inx0.313in)-1111-2016:35 ↔ 0.5inThunderHexShaft(5in(modified))-1111-2016:6
- Flush:71: 0.5inHexFlangedBearing(1.125inx0.313in)-1111-2016:36 ↔ 0.5inThunderHexShaft(5in(modified))-1111-2016:7
- Flush:72: 0.5inHexFlangedBearing(1.125inx0.313in)-1111-2016:25 ↔ 0.5inThunderHexShaft(5in(modified))-1111-2016:1
- Flush:73: 0.5inHexFlangedBearing(1.125inx0.313in)-1111-2016:33 ↔ 0.5inThunderHexShaft(5in(modified))-1111-2016:5
- Flush:74: 0.5inHexFlangedBearing(1.125inx0.313in)-1111-2016:42 ↔ 0.5inThunderHexShaft(5in(modified))-1111-2016:8
- Flush:75: 0.5inHexFlangedBearing(1.125inx0.313in)-1111-2016:40 ↔ 0.5inThunderHexShaft(5in(modified))-1111-2016:11
- Flush:76: 0.5inHexFlangedBearing(1.125inx0.313in)-1111-2016:39 ↔ 0.5inThunderHexShaft(5in(modified))-1111-2016:9
- Flush:77: 0.5inHexFlangedBearing(1.125inx0.313in)-1111-2016:41 ↔ 0.5inThunderHexShaft(5in(modified))-1111-2016:10
## Named parameters: d93_d89_d76 = 0 mm, d94_d90 = 0 mm, d103_d89_d76 = 0 mm, d104_d90 = 0 mm
